# Autodesk Inventor assembly: Ensamblaje5
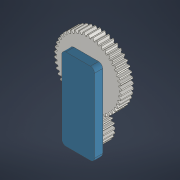
[picture p0: Inventor's stored thumbnail of the model, 180x180]
Saved by Autodesk Inventor 2022 (Build 260153000, 153)
## iProperties
Created: 2022-05-05
Part Number: Ensamblaje5
Document SubType Name: Assembly
Designer: aleon
Author: aleon
## Documents named in this file (3)
- C:\Users\aleon\OneDrive\Escritorio\Engranes\Ensamblaje5.iam
- C:\Users\aleon\OneDrive\Escritorio\Engranes\Soporte Engrane.ipt
- C:\Users\aleon\OneDrive\Escritorio\Engranes\Ensamblaje5\Design Accelerator\Engranajes rectos5.iam
## Components (2 placed, 2 different names)
1. Soporte Engrane:1 — Coincidencia:1, Coincidencia:2, Coincidencia:3, Coincidencia:4
2. Engranajes rectos:1 [sub-assembly] — Coincidencia:1, Coincidencia:2, Coincidencia:3, Coincidencia:4
## Relationships (4: Mate 4)
- Coincidencia:1 [Mate]: Soporte Engrane:1 ↔ Engranajes rectos:1
- Coincidencia:2 [Mate]: Soporte Engrane:1 ↔ Engranajes rectos:1
- Coincidencia:3 [Mate]: Soporte Engrane:1 ↔ Engranajes rectos:1
- Coincidencia:4 [Mate]: Soporte Engrane:1 ↔ Engranajes rectos:1
